# Autodesk Inventor assembly: Substructure
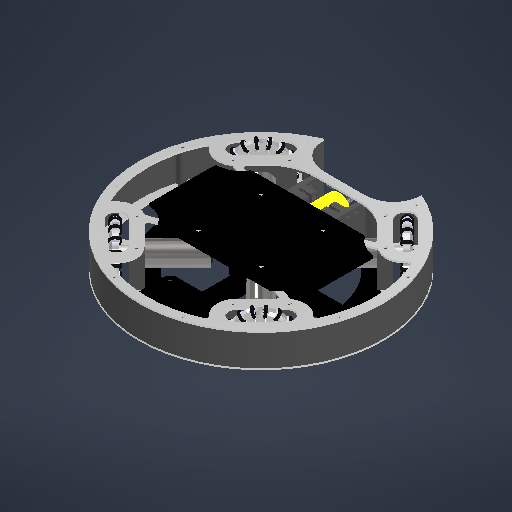
[picture p0: Inventor's stored thumbnail of the model, 512x512]
Saved by Autodesk Inventor 2025.2 (Build 292293000, 293)
## iProperties
Created: 2023-05-12
Part Number: Substructure
Document SubType Name: Assembly
Designer: Elias Braun
Author: Elias Braun
## Documents named in this file (9)
- C:\Users\EliasBraun\Nextcloud2\RoboCup2023 - WM\Substructure.iam
- C:\Users\EliasBraun\Nextcloud2\RoboCup2023 - WM\PCB\LineDedectionPCB-V1.ipt
- C:\Users\EliasBraun\Nextcloud2\RoboCup2023 - WM\CarbonRings\BottomCarbonRing.ipt
- C:\Users\EliasBraun\Nextcloud2\RoboCup2023 - WM\Motor\Drive.iam
- C:\Users\EliasBraun\Nextcloud2\RoboCup2023 - WM\Protector\Protector-WithShoot.ipt
- C:\Users\EliasBraun\Nextcloud2\RoboCup2023 - WM\Shoot\Schuss.iam
- C:\Users\EliasBraun\Nextcloud2\RoboCup2023 - WM\PCB\ShootPCB.ipt
- C:\Users\EliasBraun\Nextcloud2\RoboCup2023 - WM\CarbonRings\TopCarbonRing-WithoutClosure.ipt
- C:\Users\EliasBraun\Nextcloud2\RoboCup2023 - WM\PCB\ControllerPCB-V1.ipt
## Components (11 placed, 8 different names)
1. LineDedectionPCB-V1:1 — Mate:1, Mate:2, Mate:3
2. BottomCarbonRing:1 — Mate:1, Mate:2, Mate:3, Mate:4, Mate:5, Mate:6, Mate:7, Mate:8, Mate:9, Mate:10, Mate:11, Mate:12, Mate:13, Mate:14, Mate:15, Mate:16, Mate:17, Mate:18
3. Drive:1 [sub-assembly] — Mate:4, Mate:5, Mate:6
4. Drive:2 [sub-assembly] — Mate:7, Mate:8, Mate:9, Mate:23, Mate:24, Mate:25
5. Drive:3 [sub-assembly] — Mate:10, Mate:11, Mate:12
6. Drive:4 [sub-assembly] — Mate:13, Mate:14, Mate:15
7. Protector-WithShoot:1 — Mate:16, Mate:17, Mate:18, Mate:19, Mate:20, Mate:21, Mate:22
8. Schuss:1 [sub-assembly] — Mate:19
9. ShootPCB:1 — Mate:20, Mate:21, Mate:22
10. TopCarbonRing-WithoutClosure:1 — Mate:23, Mate:24, Mate:25, Mate:26, Mate:27, Mate:28
11. ControllerPCB-V1:1 — Mate:26, Mate:27, Mate:28
## Relationships (28: Mate 28)
- Mate:1: LineDedectionPCB-V1:1 ↔ BottomCarbonRing:1
- Mate:2: LineDedectionPCB-V1:1 ↔ BottomCarbonRing:1
- Mate:3: LineDedectionPCB-V1:1 ↔ BottomCarbonRing:1
- Mate:4: BottomCarbonRing:1 ↔ Drive:1
- Mate:5: BottomCarbonRing:1 ↔ Drive:1
- Mate:6: BottomCarbonRing:1 ↔ Drive:1
- Mate:7: BottomCarbonRing:1 ↔ Drive:2
- Mate:8: BottomCarbonRing:1 ↔ Drive:2
- Mate:9: BottomCarbonRing:1 ↔ Drive:2
- Mate:10: BottomCarbonRing:1 ↔ Drive:3
- Mate:11: BottomCarbonRing:1 ↔ Drive:3
- Mate:12: BottomCarbonRing:1 ↔ Drive:3
- Mate:13: BottomCarbonRing:1 ↔ Drive:4
- Mate:14: BottomCarbonRing:1 ↔ Drive:4
- Mate:15: BottomCarbonRing:1 ↔ Drive:4
- Mate:16: BottomCarbonRing:1 ↔ Protector-WithShoot:1
- Mate:17: BottomCarbonRing:1 ↔ Protector-WithShoot:1
- Mate:18: BottomCarbonRing:1 ↔ Protector-WithShoot:1
- Mate:19: Protector-WithShoot:1 ↔ Schuss:1
- Mate:20: Protector-WithShoot:1 ↔ ShootPCB:1
- Mate:21: Protector-WithShoot:1 ↔ ShootPCB:1
- Mate:22: Protector-WithShoot:1 ↔ ShootPCB:1
- Mate:23: Drive:2 ↔ TopCarbonRing-WithoutClosure:1
- Mate:24: Drive:2 ↔ TopCarbonRing-WithoutClosure:1
- Mate:25: Drive:2 ↔ TopCarbonRing-WithoutClosure:1
- Mate:26: TopCarbonRing-WithoutClosure:1 ↔ ControllerPCB-V1:1
- Mate:27: TopCarbonRing-WithoutClosure:1 ↔ ControllerPCB-V1:1
- Mate:28: TopCarbonRing-WithoutClosure:1 ↔ ControllerPCB-V1:1
